# Autodesk Inventor assembly: TestMerger
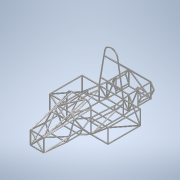
[picture p0: Inventor's stored thumbnail of the model, 180x180]
Saved by Autodesk Inventor 2021 (Build 250183000, 183)
## iProperties
Created: 2020-10-11
Part Number: TestMerger
Document SubType Name: Assembly
Designer: qv17m
_SolveAssemblyDoc: Frame Generator Solve Assembly
_Version: 25.0.0
Author: qv17m
## Documents named in this file (4)
- C:\Users\qv17m\Documents\Inventor\FSAE\RearFrame Oct 10\TestMerger.iam
- C:\Users\qv17m\Documents\Inventor\FSAE\Temp\FSAE_Frame.0007.ipt
- C:\Users\qv17m\Documents\Inventor\FSAE\RearFrame Oct 10\DesignReviewOct_10 - Copy.ipt
- C:\Users\qv17m\Documents\Inventor\FSAE\RearFrame Oct 10\TestMerger\Frame\Frame.iam
## Components (3 placed, 3 different names)
1. FSAE_Frame.0007:1 — Mate:1
2. DesignReviewOct_10 - Copy:1 — Mate:1
3. Frame:1 [sub-assembly]
## Relationships (1: Mate 1)
- Mate:1: FSAE_Frame.0007:1 ↔ DesignReviewOct_10 - Copy:1
